# Autodesk Inventor assembly: Connessione B
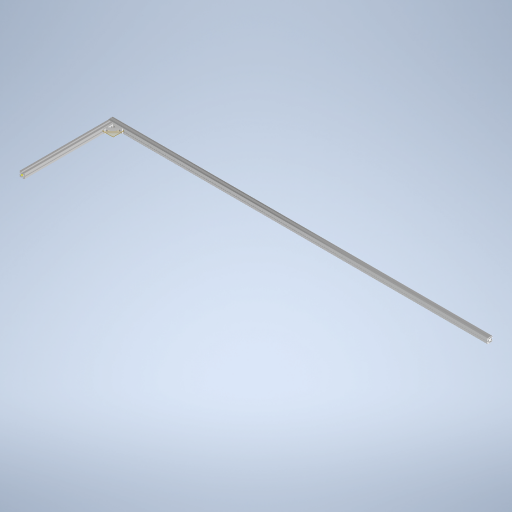
[picture p0: Inventor's stored thumbnail of the model, 512x512]
Saved by Autodesk Inventor 2023 (Build 270158000, 158)
## iProperties
Created: 2022-01-26
Part Number: Connessione B
Document SubType Name: Assembly
Designer: matte
Author: matte
## Documents named in this file (10)
- C:\Users\utente\OneDrive\Documenti\UniTN\I semestre\Connessione B.iam
- C:\Users\utente\OneDrive\Documenti\UniTN\I semestre\Mechanical Design\MDM-CyberOrto-CAD\Parker components\03-Brackets_Gussets_Plates\09-Machined Gussets\20-102.ipt
- C:\Users\utente\OneDrive\Documenti\UniTN\I semestre\Mechanical Design\MDM-CyberOrto-CAD\Parker components\02-Fasteners\10-Standard T-Nuts\20-050.ipt
- C:\Users\utente\OneDrive\Documenti\UniTN\I semestre\Mechanical Design\MDM-CyberOrto-CAD\Parker components\02-Fasteners\16-Screws\01-Metric Screws\01-Button Head\24-118-8.ipt
- C:\Users\utente\OneDrive\Documenti\UniTN\I semestre\Mechanical Design\MDM-CyberOrto-CAD\Pezzi singoli\Supporto SX.ipt
- C:\Users\utente\OneDrive\Documenti\UniTN\I semestre\Mechanical Design\MDM-CyberOrto-CAD\Pezzi singoli\10-040.ipt
- C:\Users\utente\OneDrive\Documenti\UniTN\I semestre\Mechanical Design\MDM-CyberOrto-CAD\Rack_Pinion\Rack gear scaled1.ipt
- C:\Users\utente\OneDrive\Documenti\UniTN\I semestre\Mechanical Design\MDM-CyberOrto-CAD\Parker components\02-Fasteners\16-Screws\01-Metric Screws\03-Socket Head\24-320-8SS.ipt
- C:\Users\utente\OneDrive\Documenti\UniTN\I semestre\Mechanical Design\MDM-CyberOrto-CAD\Pezzi singoli\13-106_f.ipt
- C:\Users\utente\OneDrive\Documenti\UniTN\I semestre\Mechanical Design\MDM-CyberOrto-CAD\Pezzi singoli\13-513.ipt
## Components (16 placed, 9 different names)
1. Supporto SX:2
2. 20-102:2
3. 20-050:3
4. 20-050:4
5. 24-118-8:5
6. 24-118-8:6
7. 24-118-8:7
8. 24-118-8:8
9. Rack gear scaled1:1
10. 24-320-8SS:1
11. 24-320-8SS:2
12. 13-106_f:1
13. 13-106_f:2
14. 13-513:1
15. 13-513:2
16. 10-040:2
## Relationships (37: Mate 26, Flush 11)
- [Mate]: 20-102:2 ↔ 10-040:2
- [Mate]: Supporto SX:2 ↔ 20-102:2
- [Flush]: Supporto SX:2 ↔ 20-102:2
- [Mate]: Supporto SX:2 ↔ 20-050:3
- [Mate]: 20-102:2 ↔ 20-050:3
- [Mate]: 20-102:2 ↔ 20-050:3
- [Mate]: 20-050:4 ↔ 10-040:2
- [Mate]: 20-102:2 ↔ 20-050:4
- [Mate]: 20-102:2 ↔ 20-050:4
- [Mate]: 20-102:2 ↔ 24-118-8:5
- [Mate]: 20-102:2 ↔ 24-118-8:5
- [Mate]: 20-102:2 ↔ 24-118-8:6
- [Mate]: 20-102:2 ↔ 24-118-8:6
- [Mate]: 20-102:2 ↔ 24-118-8:7
- [Mate]: 20-102:2 ↔ 24-118-8:7
- [Mate]: 20-102:2 ↔ 24-118-8:8
- [Mate]: 20-102:2 ↔ 24-118-8:8
- [Mate]: Rack gear scaled1:1 ↔ 24-320-8SS:1
- [Flush]: Rack gear scaled1:1 ↔ 24-320-8SS:1
- [Mate]: Rack gear scaled1:1 ↔ 24-320-8SS:2
- [Flush]: Rack gear scaled1:1 ↔ 24-320-8SS:2
- [Flush]: Rack gear scaled1:1 ↔ 10-040:2
- [Mate]: Rack gear scaled1:1 ↔ 10-040:2
- [Flush] (13 mm): Rack gear scaled1:1 ↔ 10-040:2
- [Flush]: 13-106_f:2 ↔ 10-040:2
- [Mate]: 13-106_f:2 ↔ 10-040:2
- [Mate]: 13-106_f:2 ↔ 10-040:2
- [Flush]: 13-106_f:1 ↔ 10-040:2
- [Mate]: 13-106_f:1 ↔ 10-040:2
- [Mate]: 13-106_f:1 ↔ 10-040:2
- [Flush]: 13-513:1 ↔ 10-040:2
- [Flush]: 13-513:2 ↔ 10-040:2
- [Mate]: 13-106_f:2 ↔ 13-513:2
- [Mate]: 13-106_f:1 ↔ 13-513:1
- [Flush]: Supporto SX:2 ↔ 10-040:2
- [Mate]: Supporto SX:2 ↔ 10-040:2
- [Flush]: Supporto SX:2 ↔ 10-040:2
## Named parameters: d495_d398_d369 = 0 mm, d496_d399_d370 = 0 mm, d497_d400_d371 = 0 mm, d498_d401_d372 = 0 mm, d51_d15 = 0 mm, d52_d16 = 0 mm, d54_d18 = 0 mm, d55_d19 = 0 mm, d56_d20 = 0 mm, d57_d21 = 0 mm, d58_d24 = 0 mm, d59_d25 = 0 mm, d60_d26 = 0 mm, d61_d27 = 0 mm, d62_d28 = 0 mm, d63_d29 = 0 mm
